# Autodesk Inventor assembly: assembl nozzle
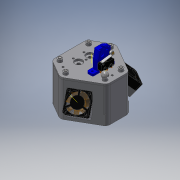
[picture p0: Inventor's stored thumbnail of the model, 180x180]
Saved by Autodesk Inventor 2016 SP1 (Build 200210100, 210)
## iProperties
Created: 2016-04-15
Part Number: assembl nozzle
Document SubType Name: Assembly
Designer: ubik
Author: ubik
## Documents named in this file (12)
- E:\GitHub\kossel-XXL\assembl nozzle.iam
- E:\GitHub\kossel-XXL\efector.ipt
- E:\GitHub\kossel-XXL\nozzel heat sink.ipt
- E:\GitHub\kossel-XXL\nozzle throat.ipt
- C:\Users\ubik\Documents\Inventor\Content Center Files\R2016\en-US\AS 1420\AS 1420 - 1973 - M4 x 8.ipt
- E:\GitHub\kossel-XXL\10mm sfere.ipt
- E:\GitHub\kossel-XXL\heated block.ipt
- E:\GitHub\kossel-XXL\nozzle.ipt
- E:\GitHub\kossel-XXL\30mm Fan.iam
- E:\GitHub\kossel-XXL\nozle mask front.ipt
- E:\GitHub\kossel-XXL\Retractable Z Probe Bracket bad.ipt
- E:\GitHub\kossel-XXL\microswitch\Microswitch_-_Omron_SS-01GL2-E.iam
## Components (21 placed, 11 different names)
1. efector:1 — Mate:5, Mate:6, Mate:7, Insert:1, Insert:2, Insert:3, Insert:4, Insert:5, Insert:6, Tangent:1, Flush:7, Mate:18, Mate:24, Mate:25, Mate:26
2. nozzel heat sink:1 — Mate:1, Mate:2, Mate:3, Mate:4, Mate:5, Mate:6, Mate:7, Mate:12, Flush:5, Mate:16, Flush:6
3. nozzle throat:1 — Mate:1, Mate:3, Mate:10
4. nozzle throat:2 — Mate:2, Mate:4, Mate:11
5. 10mm sfere:1 — Mate:9, Tangent:1
6. heated block:1 — Mate:10, Flush:3, Mate:12, Mate:13, Mate:15
7. heated block:2 — Mate:11, Flush:3, Mate:14
8. nozzle:1 — Mate:13, Flush:4, Mate:15, Mate:20
9. nozzle:2 — Mate:14, Flush:4
10. 30mm Fan:1 [sub-assembly] — Flush:5, Mate:16, Flush:6
11. nozle mask front:1 — Flush:7, Flush:9, Mate:17, Angle:1, Mate:19, Flush:11, Mate:20, Mate:21
12. 30mm Fan:2 [sub-assembly] — Mate:17, Angle:1, Mate:18, Mate:19, Flush:11
13. 30mm Fan:3 [sub-assembly] — Flush:9, Mate:21
14. Retractable Z Probe Bracket bad:1 — Mate:22, Mate:23, Mate:24, Mate:25, Mate:26
15. Microswitch_-_Omron_SS-01GL2-E:1 [sub-assembly] — Mate:22, Mate:23
16. AS 1420 - Metric M4 x 8:1 — Insert:1
17. AS 1420 - Metric M4 x 8:2 — Insert:2
18. AS 1420 - Metric M4 x 8:3 — Insert:3, Mate:9
19. AS 1420 - Metric M4 x 8:4 — Insert:4
20. AS 1420 - Metric M4 x 8:5 — Insert:5
21. AS 1420 - Metric M4 x 8:6 — Insert:6
## Relationships (40: Mate 25, Flush 7, Insert 6, Tangent 1, Angle 1)
- Mate:1: nozzel heat sink:1 ↔ nozzle throat:1
- Mate:2: nozzel heat sink:1 ↔ nozzle throat:2
- Mate:3: nozzel heat sink:1 ↔ nozzle throat:1
- Mate:4: nozzel heat sink:1 ↔ nozzle throat:2
- Mate:5: efector:1 ↔ nozzel heat sink:1
- Mate:6: efector:1 ↔ nozzel heat sink:1
- Mate:7: efector:1 ↔ nozzel heat sink:1
- Insert:1: efector:1 ↔ AS 1420 - Metric M4 x 8:1
- Insert:2: efector:1 ↔ AS 1420 - Metric M4 x 8:2
- Insert:3: efector:1 ↔ AS 1420 - Metric M4 x 8:3
- Insert:4: efector:1 ↔ AS 1420 - Metric M4 x 8:4
- Insert:5: efector:1 ↔ AS 1420 - Metric M4 x 8:5
- Insert:6: efector:1 ↔ AS 1420 - Metric M4 x 8:6
- Mate:9: 10mm sfere:1 ↔ AS 1420 - Metric M4 x 8:3
- Tangent:1: efector:1 ↔ 10mm sfere:1
- Mate:10: nozzle throat:1 ↔ heated block:1
- Mate:11: nozzle throat:2 ↔ heated block:2
- Flush:3: heated block:1 ↔ heated block:2
- Mate:12 (3 mm): nozzel heat sink:1 ↔ heated block:1
- Mate:13: heated block:1 ↔ nozzle:1
- Mate:14: heated block:2 ↔ nozzle:2
- Flush:4: nozzle:1 ↔ nozzle:2
- Mate:15 (2 mm): heated block:1 ↔ nozzle:1
- Flush:5: nozzel heat sink:1 ↔ 30mm Fan:1
- Mate:16: nozzel heat sink:1 ↔ 30mm Fan:1
- Flush:6: nozzel heat sink:1 ↔ 30mm Fan:1
- Flush:7: efector:1 ↔ nozle mask front:1
- Flush:9: nozle mask front:1 ↔ 30mm Fan:3
- Mate:17 (-15 mm): nozle mask front:1 ↔ 30mm Fan:2
- Angle:1 (45 deg): nozle mask front:1 ↔ 30mm Fan:2
- Mate:18 (10 mm): efector:1 ↔ 30mm Fan:2
- Mate:19: nozle mask front:1 ↔ 30mm Fan:2
- Flush:11: nozle mask front:1 ↔ 30mm Fan:2
- Mate:20: nozzle:1 ↔ nozle mask front:1
- Mate:21: nozle mask front:1 ↔ 30mm Fan:3
- Mate:22: Retractable Z Probe Bracket bad:1 ↔ Microswitch_-_Omron_SS-01GL2-E:1
- Mate:23: Retractable Z Probe Bracket bad:1 ↔ Microswitch_-_Omron_SS-01GL2-E:1
- Mate:24: efector:1 ↔ Retractable Z Probe Bracket bad:1
- Mate:25: efector:1 ↔ Retractable Z Probe Bracket bad:1
- Mate:26: efector:1 ↔ Retractable Z Probe Bracket bad:1
